# Autodesk Inventor assembly: BLACKBOARD
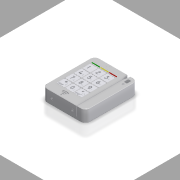
[picture p0: Inventor's stored thumbnail of the model, 180x180]
Saved by Autodesk Inventor 2014 SP2 (Build 180246200, 246)
## iProperties
Created: 2016-01-20
Document SubType Name: Assembly
Designer: Mervart
Mass: 95.1008 g
Surface Area: 961.996 cm^2
Volume: 84.9989 cm^3
Density: 1.11885 g/cm^3
LastSaveDate: 12.08.2010
Hmotnost: 0
Author: Mervart
Title: BLACKBOARD
## Documents named in this file (11)
- C:\Users\mervarto\Desktop\soutěž\3D - 1\Blackboard.iam
- C:\Users\mervarto\Desktop\soutěž\3D - 1\body.ipt
- C:\Users\mervarto\Desktop\soutěž\3D - 1\keyboard.ipt
- C:\Users\mervarto\Desktop\soutěž\3D - 1\body2.ipt
- C:\Inventor-nastaveni\Soubory obsahoveho centra\cs-CZ\CNS 4306 - AB\CNS 4306 - M2,9 x 19AB.ipt
- C:\Users\mervarto\Desktop\soutěž\3D - 1\LED green.ipt
- C:\Users\mervarto\Desktop\soutěž\3D - 1\LED yellow.ipt
- C:\Users\mervarto\Desktop\soutěž\3D - 1\LED red.ipt
- C:\Inventor-nastaveni\Soubory obsahoveho centra\cs-CZ\DIN 7991(2)\DIN 7991 - M3x8.ipt
- C:\Inventor-nastaveni\Soubory obsahoveho centra\cs-CZ\DIN 934\DIN 934 - M3 x 0,5.ipt
- C:\Users\mervarto\Desktop\soutěž\3D - 1\card.ipt
## Components (15 placed, 10 different names)
1. body:1 — Stejný směr:1, Proti sobě:1, Proti sobě:2, Stejný směr:2, Stejný směr:3, Stejný směr:4, Stejný směr:5, Rotační:3, Proti sobě:3, Proti sobě:4
2. keyboard:1 — Stejný směr:1, Proti sobě:1, Proti sobě:2
3. body2:1 — Stejný směr:2, Rotační:1, Rotační:2
4. LED green:1 — Stejný směr:3
5. LED yellow:1 — Stejný směr:4
6. LED red:1 — Stejný směr:5
7. card:1 — Proti sobě:3, Proti sobě:4
8. CNS 4306 - AB M2,9 x 19:1 — Rotační:1
9. CNS 4306 - AB M2,9 x 19:2
10. CNS 4306 - AB M2,9 x 19:3
11. CNS 4306 - AB M2,9 x 19:4
12. DIN 934 - nahrazený DIN EN 24032/28673/28674 M3:1 — Rotační:2
13. DIN 934 - nahrazený DIN EN 24032/28673/28674 M3:2
14. DIN 7991 M3x8:1 — Rotační:3
15. DIN 7991 M3x8:2
## Component patterns: (4 elements, first: CNS 4306 - AB M2,9 x 19:1), (2 elements, first: DIN 934 - nahrazený DIN EN 24032/28673/28674 M3:1), (2 elements, first: DIN 7991 M3x8:1)
## Relationships (12: Flush 5, Mate 4, RevoluteJoint 3)
- Stejný směr:1 [Flush]: body:1 ↔ keyboard:1
- Proti sobě:1 [Mate] (0.2 mm): body:1 ↔ keyboard:1
- Proti sobě:2 [Mate] (0.2 mm): body:1 ↔ keyboard:1
- Stejný směr:2 [Flush]: body:1 ↔ body2:1
- Rotační:1 [RevoluteJoint]: body2:1 ↔ CNS 4306 - AB M2,9 x 19:1
- Stejný směr:3 [Flush]: body:1 ↔ LED green:1
- Stejný směr:4 [Flush]: body:1 ↔ LED yellow:1
- Stejný směr:5 [Flush]: body:1 ↔ LED red:1
- Rotační:2 [RevoluteJoint]: body2:1 ↔ DIN 934 - nahrazený DIN EN 24032/28673/28674 M3:1
- Rotační:3 [RevoluteJoint]: body:1 ↔ DIN 7991 M3x8:1
- Proti sobě:3 [Mate]: body:1 ↔ card:1
- Proti sobě:4 [Mate]: body:1 ↔ card:1
